# Autodesk Inventor assembly: Mr.Green
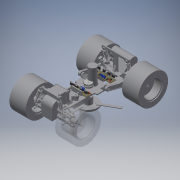
[picture p0: Inventor's stored thumbnail of the model, 180x180]
Saved by Autodesk Inventor 2019 (Build 230136000, 136)
## iProperties
Created: 2019-03-02
Part Number: Mr.Green
Document SubType Name: Assembly
Designer: alarr
Author: alarr
## Documents named in this file (17)
- C:\Users\alarr\OneDrive\Documents\Inventor\Mr.Green\Mr.Green.iam
- C:\Users\alarr\OneDrive\Documents\Inventor\Mr.Green\Back_Wheel_Drive.iam
- C:\Users\alarr\OneDrive\Documents\Inventor\Mr.Green\Wheel.iam
- C:\Users\alarr\OneDrive\Documents\Inventor\Mr.Green\Shock_Arm.ipt
- C:\Users\alarr\OneDrive\Documents\Inventor\Mr.Green\Shock_Arm_MIR.ipt
- C:\Users\alarr\OneDrive\Documents\Inventor\Mr.Green\Front_Wheel_Drive.iam
- C:\Users\alarr\OneDrive\Documents\Inventor\Mr.Green\Assembled_Cutter.iam
- C:\Users\alarr\OneDrive\Documents\Inventor\Mr.Green\Chassis.ipt
- C:\Users\alarr\OneDrive\Documents\Inventor\Mr.Green\Shock_Absorber.iam
- C:\Users\alarr\OneDrive\Documents\Inventor\Mr.Green\Shock_Absorber_MIR.iam
- C:\Users\alarr\OneDrive\Documents\Inventor\Mr.Green\Motor.ipt
- C:\Users\alarr\OneDrive\Documents\Inventor\Mr.Green\Mr.Green\Design Accelerator\Spur Gears1.iam
- C:\Users\alarr\OneDrive\Documents\Inventor\Mr.Green\Mr.Green\Design Accelerator\Shaft2.iam
- C:\Users\alarr\OneDrive\Documents\Inventor\Mr.Green\Mr.Green\Design Accelerator\Key Connection1.iam
- C:\Users\alarr\OneDrive\Documents\eagle\projects\Motor_Driver\Fusion360\Motor_Driver v44.iam
- C:\Users\alarr\OneDrive\Documents\Inventor\Mr.Green\FPGA.ipt
- C:\Users\alarr\OneDrive\Documents\Inventor\Mr.Green\Shock_Tower.ipt
## Components (20 placed, 16 different names)
1. Back_Wheel_Drive:1 [sub-assembly] — Mate:7, Mate:8, Mate:9, Mate:10, Mate:11, Mate:12, Mate:13, Mate:14, Angle:1, Mate:15, Mate:16, Angle:2, Mate:23, Flush:1, Flush:2, Mate:33
2. Shock_Arm:1 — Mate:7, Mate:8, Mate:9, Mate:26, Mate:28, Mate:53
3. Shock_Arm_MIR:1 — Mate:10, Mate:11, Mate:12, Mate:25, Mate:27
4. Wheel:1 [sub-assembly] — Mate:15, Mate:16, Angle:2
5. Wheel:2 [sub-assembly] — Mate:13, Mate:14, Angle:1
6. Front_Wheel_Drive:1 [sub-assembly] — Mate:17, Mate:18, Angle:3, Mate:19, Mate:20, Angle:4, Mate:21, Flush:2, Mate:51, Mate:54
7. Wheel:3 [sub-assembly] — Mate:17, Mate:18, Angle:3
8. Wheel:4 [sub-assembly] — Mate:19, Mate:20, Angle:4
9. Assembled_Cutter:1 [sub-assembly] — Mate:24, Mate:42, Mate:76, Mate:78
10. Chassis:1 — Flush:3, Mate:24, Mate:33, Mate:51, Mate:53, Mate:54, Mate:56, Mate:57, Mate:59, Flush:19, Flush:20, Mate:65, Mate:67, Mate:68, Mate:79
11. Shock_Absorber:1 [sub-assembly] — Mate:26, Mate:28, Mate:60
12. Shock_Absorber_MIR:1 [sub-assembly] — Mate:25, Mate:27, Mate:62
13. Motor:1 — Mate:67, Mate:68, Mate:75, Flush:24, Mate:79
14. Spur Gears:1 [sub-assembly] — Mate:38, Mate:39, Mate:52, Angle:13, Mate:75, Flush:24
15. Shaft:1 [sub-assembly] — Mate:38, Mate:39, Mate:42, Angle:13, Mate:76, Angle:16, Mate:78, Flush:25, Angle:17, Mate:80
16. Key Connection:1 [sub-assembly] — Mate:52, Flush:25, Angle:17, Mate:80
17. Motor_Driver v44:1 [sub-assembly] — Mate:56, Mate:57, Mate:66
18. FPGA:1 — Mate:65
19. Motor_Driver v44:2 [sub-assembly] — Mate:66, Mate:59
20. Shock_Tower:1 — Flush:19, Mate:60, Flush:20, Mate:62
## Relationships (58: Mate 44, Angle 7, Flush 7)
- Mate:7: Back_Wheel_Drive:1 ↔ Shock_Arm:1
- Mate:8: Back_Wheel_Drive:1 ↔ Shock_Arm:1
- Mate:9: Back_Wheel_Drive:1 ↔ Shock_Arm:1
- Mate:10: Back_Wheel_Drive:1 ↔ Shock_Arm_MIR:1
- Mate:11: Back_Wheel_Drive:1 ↔ Shock_Arm_MIR:1
- Mate:12: Back_Wheel_Drive:1 ↔ Shock_Arm_MIR:1
- Mate:13: Back_Wheel_Drive:1 ↔ Wheel:2
- Mate:14: Back_Wheel_Drive:1 ↔ Wheel:2
- Angle:1 (0 deg): Back_Wheel_Drive:1 ↔ Wheel:2
- Mate:15: Back_Wheel_Drive:1 ↔ Wheel:1
- Mate:16: Back_Wheel_Drive:1 ↔ Wheel:1
- Angle:2 (0 deg): Back_Wheel_Drive:1 ↔ Wheel:1
- Mate:17: Front_Wheel_Drive:1 ↔ Wheel:3
- Mate:18: Front_Wheel_Drive:1 ↔ Wheel:3
- Angle:3 (0 deg): Front_Wheel_Drive:1 ↔ Wheel:3
- Mate:19: Front_Wheel_Drive:1 ↔ Wheel:4
- Mate:20: Front_Wheel_Drive:1 ↔ Wheel:4
- Angle:4 (0 deg): Front_Wheel_Drive:1 ↔ Wheel:4
- Mate:21: Front_Wheel_Drive:1
- Mate:22
- Mate:23: Back_Wheel_Drive:1
- Flush:1: Back_Wheel_Drive:1
- Flush:2: Back_Wheel_Drive:1 ↔ Front_Wheel_Drive:1
- Flush:3 (15.24 mm): Chassis:1
- Mate:24: Assembled_Cutter:1 ↔ Chassis:1
- Mate:25: Shock_Arm_MIR:1 ↔ Shock_Absorber_MIR:1
- Mate:26: Shock_Arm:1 ↔ Shock_Absorber:1
- Mate:27: Shock_Arm_MIR:1 ↔ Shock_Absorber_MIR:1
- Mate:28: Shock_Arm:1 ↔ Shock_Absorber:1
- Mate:33: Back_Wheel_Drive:1 ↔ Chassis:1
- Mate:38: Spur Gears:1 ↔ Shaft:1
- Mate:39: Spur Gears:1 ↔ Shaft:1
- Mate:42: Assembled_Cutter:1 ↔ Shaft:1
- Mate:51: Front_Wheel_Drive:1 ↔ Chassis:1
- Mate:52: Spur Gears:1 ↔ Key Connection:1
- Mate:53: Shock_Arm:1 ↔ Chassis:1
- Mate:54: Front_Wheel_Drive:1 ↔ Chassis:1
- Mate:56: Chassis:1 ↔ Motor_Driver v44:1
- Mate:57: Chassis:1 ↔ Motor_Driver v44:1
- Mate:66: Motor_Driver v44:1 ↔ Motor_Driver v44:2
- Mate:59: Chassis:1 ↔ Motor_Driver v44:2
- Flush:19: Chassis:1 ↔ Shock_Tower:1
- Mate:60: Shock_Absorber:1 ↔ Shock_Tower:1
- Flush:20: Chassis:1 ↔ Shock_Tower:1
- Mate:62: Shock_Absorber_MIR:1 ↔ Shock_Tower:1
- Mate:65: Chassis:1 ↔ FPGA:1
- Mate:67: Chassis:1 ↔ Motor:1
- Mate:68: Chassis:1 ↔ Motor:1
- Angle:13 (176.5385 deg): Spur Gears:1 ↔ Shaft:1
- Mate:75: Motor:1 ↔ Spur Gears:1
- Flush:24: Motor:1 ↔ Spur Gears:1
- Mate:76: Assembled_Cutter:1 ↔ Shaft:1
- Angle:16 (0 deg): Shaft:1
- Mate:78: Assembled_Cutter:1 ↔ Shaft:1
- Mate:79: Chassis:1 ↔ Motor:1
- Flush:25: Shaft:1 ↔ Key Connection:1
- Angle:17 (0 deg): Shaft:1 ↔ Key Connection:1
- Mate:80: Shaft:1 ↔ Key Connection:1
